# Autodesk Inventor assembly: McCrea_RUKA_Walle
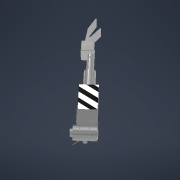
[picture p0: Inventor's stored thumbnail of the model, 180x180]
Saved by Autodesk Inventor 2022 (Build 260153000, 153)
## iProperties
Created: 2022-01-25
Part Number: McCrea_RUKA_Walle
Document SubType Name: Assembly
Designer: Lukas
Author: Lukas
## Documents named in this file (7)
- C:\Users\Lukas\Desktop\ard\3D\Walle\FINAL\lukas\McCrea_RUKA_Walle.iam
- C:\Users\Lukas\Desktop\ard\3D\Walle\FINAL\lukas\McCrea_rameno_Walle.ipt
- C:\Users\Lukas\Desktop\ard\3D\Walle\FINAL\lukas\McCrea_paza_Walle.ipt
- C:\Users\Lukas\Desktop\ard\3D\Walle\FINAL\lukas\McCrea_wrist_Walle.ipt
- C:\Users\Lukas\Desktop\ard\3D\Walle\FINAL\lukas\McCrea_arm-connector_Walle.ipt
- C:\Users\Lukas\Desktop\ard\3D\Walle\FINAL\lukas\McCrea_finger_Walle.ipt
- C:\Users\Lukas\Desktop\ard\3D\Walle\FINAL\lukas\McCrea_finger2_Walle.ipt
## Components (6 placed, 6 different names)
1. McCrea_rameno_Walle:1 — Cylindrical:1, Flush:1
2. McCrea_paza_Walle:1 — Cylindrical:1, Rigid:1, Flush:1
3. McCrea_wrist_Walle:1 — Rigid:1, Mate:6, Mate:7
4. McCrea_arm-connector_Walle:1 — Mate:1, Mate:2, Mate:3, Mate:4, Mate:5, Mate:6, Mate:7
5. McCrea_finger_Walle:1 — Mate:3, Mate:4, Mate:5
6. McCrea_finger2_Walle:1 — Mate:1, Mate:2
## Relationships (10: Mate 7, CylindricalJoint 1, WeldJoint 1, Flush 1)
- Cylindrical:1: McCrea_rameno_Walle:1 ↔ McCrea_paza_Walle:1
- Rigid:1 [WeldJoint]: McCrea_paza_Walle:1 ↔ McCrea_wrist_Walle:1
- Flush:1: McCrea_rameno_Walle:1 ↔ McCrea_paza_Walle:1
- Mate:1: McCrea_arm-connector_Walle:1 ↔ McCrea_finger2_Walle:1
- Mate:2: McCrea_arm-connector_Walle:1 ↔ McCrea_finger2_Walle:1
- Mate:3: McCrea_arm-connector_Walle:1 ↔ McCrea_finger_Walle:1
- Mate:4: McCrea_arm-connector_Walle:1 ↔ McCrea_finger_Walle:1
- Mate:5: McCrea_arm-connector_Walle:1 ↔ McCrea_finger_Walle:1
- Mate:6: McCrea_wrist_Walle:1 ↔ McCrea_arm-connector_Walle:1
- Mate:7: McCrea_wrist_Walle:1 ↔ McCrea_arm-connector_Walle:1
